# Autodesk Inventor assembly: Цепной привод2_MIR2
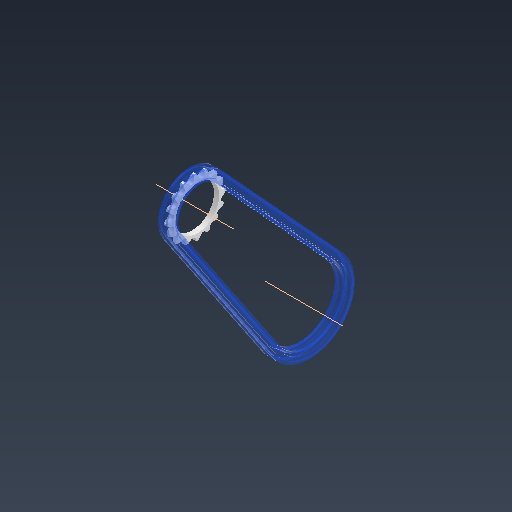
[picture p0: Inventor's stored thumbnail of the model, 512x512]
Saved by Autodesk Inventor 2025 (Build 290162000, 162)
## iProperties
Created: 2024-09-18
Part Number: Цепной привод2_MIR2
Document SubType Name: Assembly
Designer: GameHD
Author: GameHD
## Documents named in this file (4)
- C:\Users\GameHD\Desktop\Phantom 16950\Цепной привод2_MIR2.iam
- C:\Users\GameHD\Desktop\Phantom 16950\Цепь роликовая2_MIR3.ipt
- C:\Users\GameHD\Desktop\Phantom 16950\Звездочка роликовой цепи12_MIR3.ipt
- C:\Users\GameHD\Desktop\Phantom 16950\Звездочка роликовой цепи22_MIR3.ipt
## Components (3 placed, 3 different names)
1. Цепь роликовая2_MIR3:1 — Совмещение:1, Заподлицо:1, Совмещение:4, Совмещение:3, Заподлицо:2
2. Звездочка роликовой цепи12_MIR3:1 — Совмещение:1, Заподлицо:1, ЗубчПер:1
3. Звездочка роликовой цепи22_MIR3:1 — Совмещение:4, Совмещение:3, Заподлицо:2, ЗубчПер:1
## Relationships (6: Mate 3, Flush 2, RelateRotation 1)
- Совмещение:1 [Mate]: Цепь роликовая2_MIR3:1 ↔ Звездочка роликовой цепи12_MIR3:1
- Заподлицо:1 [Flush]: Цепь роликовая2_MIR3:1 ↔ Звездочка роликовой цепи12_MIR3:1
- Совмещение:4 [Mate]: Цепь роликовая2_MIR3:1 ↔ Звездочка роликовой цепи22_MIR3:1
- Совмещение:3 [Mate]: Цепь роликовая2_MIR3:1 ↔ Звездочка роликовой цепи22_MIR3:1
- Заподлицо:2 [Flush]: Цепь роликовая2_MIR3:1 ↔ Звездочка роликовой цепи22_MIR3:1
- ЗубчПер:1 [RelateRotation] (0.6667 ul): Звездочка роликовой цепи12_MIR3:1 ↔ Звездочка роликовой цепи22_MIR3:1
